# Autodesk Inventor assembly: back tire assembly ver.
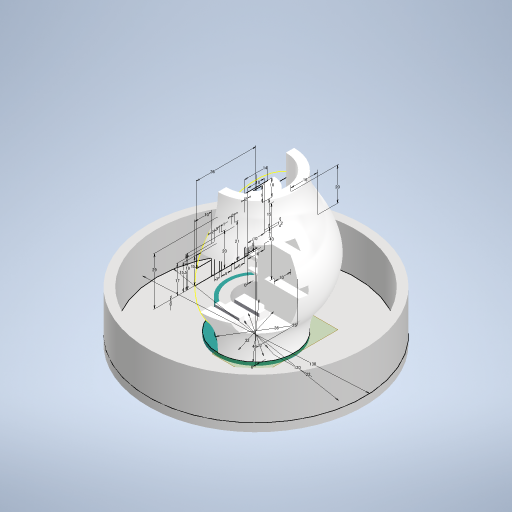
[picture p0: Inventor's stored thumbnail of the model, 512x512]
Saved by Autodesk Inventor 2023 (Build 270158000, 158)
## iProperties
Created: 2022-11-06
Part Number: back tire assembly ver.
Document SubType Name: Assembly
Designer: RM206user
Author: RM206user
## Documents named in this file (4)
- C:\Users\RM206user\Desktop\cansat\tanekonsat2022_runback\machinary\body\tire assembly\back tire assembly ver..iam
- C:\Users\RM206user\Desktop\cansat\tanekonsat2022_runback\machinary\body\body back\back moter middle tire ver\back moter middle tire lemon shape.ipt
- C:\Users\RM206user\Desktop\cansat\tanekonsat2022_runback\machinary\parts\bush.ipt
- C:\Users\RM206user\Desktop\cansat\tanekonsat2022_runback\machinary\parts\tire\tire out130 in 22 5mm inward.ipt
## Components (3 placed, 3 different names)
1. body moter middle:1 — メイト:4, メイト:5
2. bush:1 — メイト:1, メイト:2, メイト:3
3. tire out130 in 22 5mm inward:1 — メイト:1, メイト:2, メイト:3, メイト:4, メイト:5
## Relationships (5: Mate 5)
- メイト:1 [Mate]: bush:1 ↔ tire out130 in 22 5mm inward:1
- メイト:2 [Mate]: bush:1 ↔ tire out130 in 22 5mm inward:1
- メイト:3 [Mate]: bush:1 ↔ tire out130 in 22 5mm inward:1
- メイト:4 [Mate]: body moter middle:1 ↔ tire out130 in 22 5mm inward:1
- メイト:5 [Mate]: body moter middle:1 ↔ tire out130 in 22 5mm inward:1
